# Autodesk Inventor assembly: T-Metal-Brace
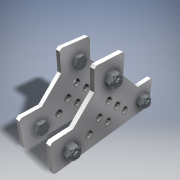
[picture p0: Inventor's stored thumbnail of the model, 180x180]
Saved by Autodesk Inventor 2017.3 (Build 213256000, 256)
## iProperties
Created: 2018-01-05
Part Number: T-Metal-Brace
Document SubType Name: Assembly
Designer: pranav
Author: pranav
## iProperties of the stored document REV-41-1359 Simple.ipt
Created: 2017-04-10
Part Number: REV-41-1359 Simple
Material: Generic
Document SubType Name: Modeling
Designer: pranav
Density: 1 g/cm^3
Appearance: Default
Sending System: Autodesk Translation Framework v5.2.0.2920
Preprocessor: ST-DEVELOPER v16.5
Title: E:/Dropbox/REV Robotics/STEP Files/REV-41-1359 Simple.step
## iProperties of the stored document REV-41-1361 Simple.ipt
Created: 2017-04-10
Part Number: REV-41-1361 Simple
Material: Generic
Document SubType Name: Modeling
Designer: pranav
Density: 1 g/cm^3
Appearance: Default
Sending System: Autodesk Translation Framework v5.2.0.2920
Preprocessor: ST-DEVELOPER v16.5
Title: E:/Dropbox/REV Robotics/STEP Files/REV-41-1361 Simple.step
## iProperties of the stored document REV-41-1025.ipt
Created: 2015-08-20
Part Number: REV-41-1025
Material: Generic
Description: STEP AP214
Document SubType Name: Modeling
Designer: pranav
Density: 1 g/cm^3
Appearance: Default
Sending System: SolidWorks 2014
Preprocessor: SwSTEP 2.0
Title: REV-41-1025_10mm.STEP
Revision Number: ANY
## Documents named in this file (7)
- **C:\Users\pranav\Documents\Inventor\REV-Robot-CAD\T-Metal-Brace.iam*LocalDocs*xGj13zqrn0cc1eb4fNxz303nlUe*REV-41-1359 Simple.ipt
- **C:\Users\pranav\Documents\Inventor\REV-Robot-CAD\T-Metal-Brace.iam*LocalDocs*x3k11kj41E41kex4tLbl0bz4sQg*REV-41-1361 Simple.ipt
- **C:\Users\pranav\Documents\Inventor\REV-Robot-CAD\T-Metal-Brace.iam*LocalDocs*xMadpayvtVsxeeu0e1qszr2ay5g*REV-41-1025.ipt
- C:\Users\pranav\Documents\Inventor\REV-Robot-CAD\T-Metal-Brace.iam
- C:\Users\pranav\Documents\Inventor\REV-Robot-CAD\REV Robotics\REV Robotics CAD\REV-41-1025.STEP
- C:\Users\pranav\Documents\Inventor\REV-Robot-CAD\REV Robotics\REV Robotics CAD\REV-41-1359 Simple.step
- C:\Users\pranav\Documents\Inventor\REV-Robot-CAD\REV Robotics\REV Robotics CAD\REV-41-1361 Simple.step
## Components (14 placed, 3 different names)
1. REV-41-1025:1 — Mate:11, Mate:13, Mate:15, Mate:16, Mate:18, Mate:20
2. REV-41-1025:2 — Mate:5, Mate:7, Mate:9, Mate:22, Mate:23, Mate:24
3. REV-41-1359 Simple:1 — Mate:11, Mate:19
4. REV-41-1359 Simple:2 — Mate:13, Mate:21
5. REV-41-1359 Simple:3 — Mate:15, Mate:17
6. REV-41-1359 Simple:4 — Mate:9, Mate:26
7. REV-41-1359 Simple:5 — Mate:5, Mate:25
8. REV-41-1359 Simple:6 — Mate:7, Mate:27
9. REV-41-1361 Simple:1 — Mate:20, Mate:21
10. REV-41-1361 Simple:2 — Mate:23, Mate:25
11. REV-41-1361 Simple:3 — Mate:22, Mate:26
12. REV-41-1361 Simple:4 — Mate:16, Mate:17
13. REV-41-1361 Simple:5 — Mate:24, Mate:27
14. REV-41-1361 Simple:6 — Mate:18, Mate:19
## Relationships (18: Mate 18)
- Mate:5: REV-41-1025:2 ↔ REV-41-1359 Simple:5
- Mate:7: REV-41-1025:2 ↔ REV-41-1359 Simple:6
- Mate:9: REV-41-1025:2 ↔ REV-41-1359 Simple:4
- Mate:11: REV-41-1025:1 ↔ REV-41-1359 Simple:1
- Mate:13: REV-41-1025:1 ↔ REV-41-1359 Simple:2
- Mate:15: REV-41-1025:1 ↔ REV-41-1359 Simple:3
- Mate:16: REV-41-1025:1 ↔ REV-41-1361 Simple:4
- Mate:17: REV-41-1359 Simple:3 ↔ REV-41-1361 Simple:4
- Mate:18: REV-41-1025:1 ↔ REV-41-1361 Simple:6
- Mate:19: REV-41-1359 Simple:1 ↔ REV-41-1361 Simple:6
- Mate:20: REV-41-1025:1 ↔ REV-41-1361 Simple:1
- Mate:21: REV-41-1359 Simple:2 ↔ REV-41-1361 Simple:1
- Mate:22: REV-41-1025:2 ↔ REV-41-1361 Simple:3
- Mate:23: REV-41-1025:2 ↔ REV-41-1361 Simple:2
- Mate:24: REV-41-1025:2 ↔ REV-41-1361 Simple:5
- Mate:25: REV-41-1359 Simple:5 ↔ REV-41-1361 Simple:2
- Mate:26: REV-41-1359 Simple:4 ↔ REV-41-1361 Simple:3
- Mate:27: REV-41-1359 Simple:6 ↔ REV-41-1361 Simple:5
